# Autodesk Inventor assembly: YAxisMotorRight
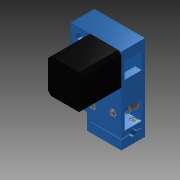
[picture p0: Inventor's stored thumbnail of the model, 180x180]
Saved by Autodesk Inventor 2015 SP1 (Build 190203100, 203)
## iProperties
Created: 2014-08-15
Part Number: YAxisMotorRight
Document SubType Name: Assembly
Designer: Jack
Mass: 234.103 g
Surface Area: 671.388 cm^2
Volume: 179.31 cm^3
Density: 1.30558 g/cm^3
Author: Jack
Title: Y Motor Right
## Documents named in this file (15)
- C:\Users\Jack\ownCloud\Projects\CrossBot\InventorModel\YAxis\YAxisMotorRight.iam
- C:\Users\Jack\ownCloud\Projects\CrossBot\InventorModel\YAxis\YAxisMotor\YMotorBlockRight.ipt
- C:\Users\Jack\ownCloud\Projects\CrossBot\InventorModel\YAxis\YAxisMotor\YMotorCapRight.ipt
- C:\Users\Jack\ownCloud\Projects\CrossBot\InventorModel\Hardware\Bolts\SHCS\SHCS4\SHCS4x30.ipt
- C:\Users\Jack\ownCloud\Projects\CrossBot\InventorModel\Hardware\Bolts\SHCS\SHCS3\SHCS3x8.ipt
- C:\Users\Jack\ownCloud\Projects\CrossBot\InventorModel\Hardware\Bearing\BearingRadialBall\BearingRadialBallF624zz.ipt
- C:\Users\Jack\ownCloud\Projects\CrossBot\InventorModel\Hardware\Wahsers\M4Washer.ipt
- C:\Users\Jack\ownCloud\Projects\CrossBot\InventorModel\Hardware\Nuts\Nut4.ipt
- C:\Users\Jack\ownCloud\Projects\CrossBot\InventorModel\YAxis\YAxisBearingSpacer.ipt
- C:\Users\Jack\ownCloud\Projects\CrossBot\InventorModel\Electronics\Motors\StepperMotorNema17x48mm.ipt
- C:\Users\Jack\ownCloud\Projects\CrossBot\InventorModel\Hardware\Belt\GT2Idler.iam
- C:\Users\Jack\ownCloud\Projects\CrossBot\InventorModel\YAxis\YAxisBeltIdlerSpacer.ipt
- C:\Users\Jack\ownCloud\Projects\CrossBot\InventorModel\Hardware\Bolts\FHS\FHS4\FHS4x8.ipt
- C:\Users\Jack\ownCloud\Projects\CrossBot\InventorModel\Hardware\Bolts\SHCS\SHCS4\SHCS4x8.ipt
- C:\Users\Jack\ownCloud\Projects\CrossBot\InventorModel\Hardware\Bolts\SHCS\SHCS4\SHCS4x14.ipt
## Components (39 placed, 14 different names)
1. YMotorBlockRight:1 — Mate:5, Flush:3, Mate:4, Mate:1, Mate:10, Mate:7, Mate:9, Mate:8, Mate:18, Mate:12, Mate:16, Mate:13, Mate:17, Mate:14, Mate:15, Mate:11, Mate:48, Angle:1, Mate:50, Mate:52, Angle:3, Angle:2, Slider:2, Mate:74, Mate:76, Mate:80, Mate:84, Mate:94, Mate:95, Mate:96, Mate:101, Mate:109, Mate:110, Flush:4, Mate:111, Mate:112, Mate:113, Mate:114, Mate:115, Flush:5, Angle:4, Angle:5, Angle:6, Angle:7, Mate:124, Mate:125, Mate:126, Mate:127, Mate:128, Mate:129, Mate:130, Mate:131
2. YMotorCapRight:1 — Mate:1, Mate:132, Mate:133, Mate:134, Mate:135, Mate:136, Mate:137
3. YAxisBearingSpacer:2 — Mate:83, Mate:84
4. YAxisBearingSpacer:3 — Mate:79, Mate:80
5. StepperMotorNema17x48mm:1 — Mate:94, Mate:95, Mate:96
6. GT2Idler:1 [sub-assembly] — Mate:102, Mate:116, Mate:117
7. YAxisBeltIdlerSpacer:1 — Mate:107, Mate:108, Mate:109
8. SHCS4x14:1 — Mate:129, Mate:133, Mate:139
9. SHCS4x14:2 — Mate:130, Mate:134, Mate:136, Mate:140
10. SHCS4x14:3 — Mate:128, Mate:132, Mate:138
11. SHCS4x14:4 — Mate:131, Mate:135, Mate:137, Mate:141
12. BearingRadialBallF624zz:1 — Mate:24, Mate:23, Mate:26, Mate:25
13. BearingRadialBallF624zz:2 — Mate:24, Mate:23, Mate:28, Mate:27
14. BearingRadialBallF624zz:5 — Mate:40, Mate:39, Mate:42, Mate:41
15. BearingRadialBallF624zz:6 — Mate:40, Mate:39, Mate:44, Mate:43
16. M4Washer:3 — Mate:37, Mate:101, Mate:117
17. M4Washer:5 — Mate:45, Mate:42, Mate:41, Mate:76
18. Nut4:3 — Mate:52, Angle:3, Mate:51
19. Nut4:2 — Mate:50, Mate:49, Angle:2
20. Nut4:1 — Mate:48, Angle:1, Mate:47
21. M4Washer:6 — Mate:44, Mate:43
22. M4Washer:4 — Mate:105, Mate:116
23. M4Washer:2 — Mate:29, Mate:28, Mate:27
24. M4Washer:1 — Mate:26, Mate:25, Mate:74
25. SHCS4x30:2 — Mate:9, Mate:8, Mate:29, Mate:47, Mate:79
26. SHCS4x30:1 — Mate:10, Mate:7, Mate:37, Mate:49, Mate:102, Mate:105, Mate:107, Mate:108
27. SHCS4x30:3 — Mate:45, Mate:51, Slider:2, Mate:83
28. FHS4x8:1 — Mate:110, Flush:4
29. SHCS4x8:1 — Mate:111, Mate:112
30. SHCS4x8:2 — Mate:113, Mate:114
31. FHS4x8:2 — Mate:115, Flush:5
32. SHCS3x8:1 — Mate:18, Mate:12
33. SHCS3x8:4 — Mate:15, Mate:11
34. SHCS3x8:3 — Mate:17, Mate:14
35. SHCS3x8:2 — Mate:16, Mate:13
36. Nut4:4 — Angle:7, Mate:127, Mate:140
37. Nut4:5 — Angle:4, Mate:126, Mate:141
38. Nut4:7 — Angle:6, Mate:125, Mate:138
39. Nut4:6 — Angle:5, Mate:124, Mate:139
## Relationships (88: Mate 78, Angle 7, Flush 2, TranslationJoint 1)
- Mate:5: YMotorBlockRight:1
- Flush:3 [Mate]: YMotorBlockRight:1
- Mate:4: YMotorBlockRight:1
- Mate:1: YMotorBlockRight:1 ↔ YMotorCapRight:1
- Mate:10: YMotorBlockRight:1 ↔ SHCS4x30:1
- Mate:7: YMotorBlockRight:1 ↔ SHCS4x30:1
- Mate:9: YMotorBlockRight:1 ↔ SHCS4x30:2
- Mate:8: YMotorBlockRight:1 ↔ SHCS4x30:2
- Mate:18: YMotorBlockRight:1 ↔ SHCS3x8:1
- Mate:12: YMotorBlockRight:1 ↔ SHCS3x8:1
- Mate:16: YMotorBlockRight:1 ↔ SHCS3x8:2
- Mate:13: YMotorBlockRight:1 ↔ SHCS3x8:2
- Mate:17: YMotorBlockRight:1 ↔ SHCS3x8:3
- Mate:14: YMotorBlockRight:1 ↔ SHCS3x8:3
- Mate:15: YMotorBlockRight:1 ↔ SHCS3x8:4
- Mate:11: YMotorBlockRight:1 ↔ SHCS3x8:4
- Mate:24: BearingRadialBallF624zz:1 ↔ BearingRadialBallF624zz:2
- Mate:23: BearingRadialBallF624zz:1 ↔ BearingRadialBallF624zz:2
- Mate:26: BearingRadialBallF624zz:1 ↔ M4Washer:1
- Mate:25: BearingRadialBallF624zz:1 ↔ M4Washer:1
- Mate:29: M4Washer:2 ↔ SHCS4x30:2
- Mate:28: BearingRadialBallF624zz:2 ↔ M4Washer:2
- Mate:27: BearingRadialBallF624zz:2 ↔ M4Washer:2
- Mate:37: M4Washer:3 ↔ SHCS4x30:1
- Mate:40: BearingRadialBallF624zz:5 ↔ BearingRadialBallF624zz:6
- Mate:39: BearingRadialBallF624zz:5 ↔ BearingRadialBallF624zz:6
- Mate:45: M4Washer:5 ↔ SHCS4x30:3
- Mate:42: BearingRadialBallF624zz:5 ↔ M4Washer:5
- Mate:41: BearingRadialBallF624zz:5 ↔ M4Washer:5
- Mate:44: BearingRadialBallF624zz:6 ↔ M4Washer:6
- Mate:43: BearingRadialBallF624zz:6 ↔ M4Washer:6
- Mate:48: YMotorBlockRight:1 ↔ Nut4:1
- Angle:1 (0 deg): YMotorBlockRight:1 ↔ Nut4:1
- Mate:47: Nut4:1 ↔ SHCS4x30:2
- Mate:50: YMotorBlockRight:1 ↔ Nut4:2
- Mate:49: Nut4:2 ↔ SHCS4x30:1
- Mate:52: YMotorBlockRight:1 ↔ Nut4:3
- Angle:3 (0 deg): YMotorBlockRight:1 ↔ Nut4:3
- Mate:51: Nut4:3 ↔ SHCS4x30:3
- Angle:2 (0 deg): YMotorBlockRight:1 ↔ Nut4:2
- Slider:2 [TranslationJoint]: YMotorBlockRight:1 ↔ SHCS4x30:3
- Mate:74: YMotorBlockRight:1 ↔ M4Washer:1
- Mate:76: YMotorBlockRight:1 ↔ M4Washer:5
- Mate:79: YAxisBearingSpacer:3 ↔ SHCS4x30:2
- Mate:80: YMotorBlockRight:1 ↔ YAxisBearingSpacer:3
- Mate:83: YAxisBearingSpacer:2 ↔ SHCS4x30:3
- Mate:84: YMotorBlockRight:1 ↔ YAxisBearingSpacer:2
- Mate:94: YMotorBlockRight:1 ↔ StepperMotorNema17x48mm:1
- Mate:95: YMotorBlockRight:1 ↔ StepperMotorNema17x48mm:1
- Mate:96: YMotorBlockRight:1 ↔ StepperMotorNema17x48mm:1
- Mate:101: YMotorBlockRight:1 ↔ M4Washer:3
- Mate:102: GT2Idler:1 ↔ SHCS4x30:1
- Mate:105: M4Washer:4 ↔ SHCS4x30:1
- Mate:107: YAxisBeltIdlerSpacer:1 ↔ SHCS4x30:1
- Mate:108: YAxisBeltIdlerSpacer:1 ↔ SHCS4x30:1
- Mate:109: YMotorBlockRight:1 ↔ YAxisBeltIdlerSpacer:1
- Mate:110: YMotorBlockRight:1 ↔ FHS4x8:1
- Flush:4: YMotorBlockRight:1 ↔ FHS4x8:1
- Mate:111: YMotorBlockRight:1 ↔ SHCS4x8:1
- Mate:112: YMotorBlockRight:1 ↔ SHCS4x8:1
- Mate:113: YMotorBlockRight:1 ↔ SHCS4x8:2
- Mate:114: YMotorBlockRight:1 ↔ SHCS4x8:2
- Mate:115: YMotorBlockRight:1 ↔ FHS4x8:2
- Flush:5: YMotorBlockRight:1 ↔ FHS4x8:2
- Mate:116: GT2Idler:1 ↔ M4Washer:4
- Mate:117: GT2Idler:1 ↔ M4Washer:3
- Angle:4 (0 deg): YMotorBlockRight:1 ↔ Nut4:5
- Angle:5 (0 deg): YMotorBlockRight:1 ↔ Nut4:6
- Angle:6 (0 deg): YMotorBlockRight:1 ↔ Nut4:7
- Angle:7 (0 deg): YMotorBlockRight:1 ↔ Nut4:4
- Mate:124: YMotorBlockRight:1 ↔ Nut4:6
- Mate:125: YMotorBlockRight:1 ↔ Nut4:7
- Mate:126: YMotorBlockRight:1 ↔ Nut4:5
- Mate:127: YMotorBlockRight:1 ↔ Nut4:4
- Mate:128: YMotorBlockRight:1 ↔ SHCS4x14:3
- Mate:129: YMotorBlockRight:1 ↔ SHCS4x14:1
- Mate:130: YMotorBlockRight:1 ↔ SHCS4x14:2
- Mate:131: YMotorBlockRight:1 ↔ SHCS4x14:4
- Mate:132: YMotorCapRight:1 ↔ SHCS4x14:3
- Mate:133: YMotorCapRight:1 ↔ SHCS4x14:1
- Mate:134: YMotorCapRight:1 ↔ SHCS4x14:2
- Mate:135: YMotorCapRight:1 ↔ SHCS4x14:4
- Mate:136: YMotorCapRight:1 ↔ SHCS4x14:2
- Mate:137: YMotorCapRight:1 ↔ SHCS4x14:4
- Mate:138: SHCS4x14:3 ↔ Nut4:7
- Mate:139: SHCS4x14:1 ↔ Nut4:6
- Mate:140: SHCS4x14:2 ↔ Nut4:4
- Mate:141: SHCS4x14:4 ↔ Nut4:5
